# Autodesk Inventor assembly: CAJA_FUENTE_ENSAMBLE
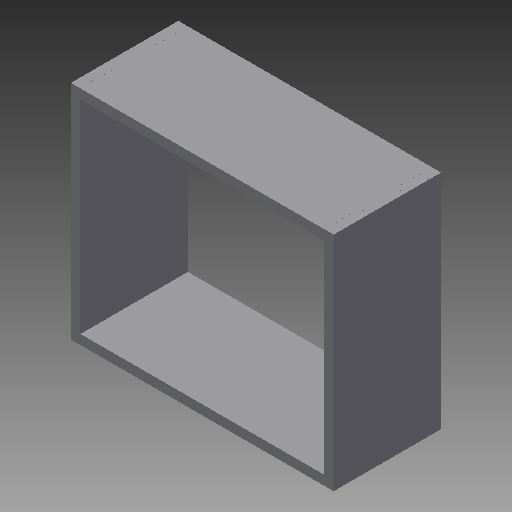
[picture p0: Inventor's stored thumbnail of the model, 512x512]
Saved by Autodesk Inventor 2018 (Build 220112000, 112)
## iProperties
Created: 2018-03-06
Part Number: CAJA_FUENTE_ENSAMBLE
Document SubType Name: Assembly
Designer: isai
Author: isai
## Documents named in this file (4)
- C:\Users\isai\Documents\GitHub\caja-reductora-II\CAJA_FUENTE_ENSAMBLE.iam
- C:\Users\isai\Documents\GitHub\caja-reductora-II\FUENTE 1.ipt
- C:\Users\isai\Documents\GitHub\caja-reductora-II\FUENTE 2.ipt
- C:\Users\isai\Documents\GitHub\caja-reductora-II\FUENTE 3.ipt
## Components (4 placed, 3 different names)
1. FUENTE 1:1 — Flush:1, Mate:1, Flush:2
2. FUENTE 2:1 — Mate:3, Flush:4, Flush:5
3. FUENTE 3:1 — Flush:1, Mate:1, Flush:2, Mate:2, Flush:3, Flush:6
4. FUENTE 1:2 — Mate:2, Flush:3, Mate:3, Flush:4, Flush:5, Flush:6
## Relationships (9: Flush 6, Mate 3)
- Flush:1: FUENTE 1:1 ↔ FUENTE 3:1
- Mate:1: FUENTE 1:1 ↔ FUENTE 3:1
- Flush:2: FUENTE 1:1 ↔ FUENTE 3:1
- Mate:2: FUENTE 3:1 ↔ FUENTE 1:2
- Flush:3: FUENTE 3:1 ↔ FUENTE 1:2
- Mate:3: FUENTE 2:1 ↔ FUENTE 1:2
- Flush:4: FUENTE 2:1 ↔ FUENTE 1:2
- Flush:5: FUENTE 2:1 ↔ FUENTE 1:2
- Flush:6: FUENTE 3:1 ↔ FUENTE 1:2
